# Autodesk Inventor assembly: 110033226_iam_10_角落碉堡
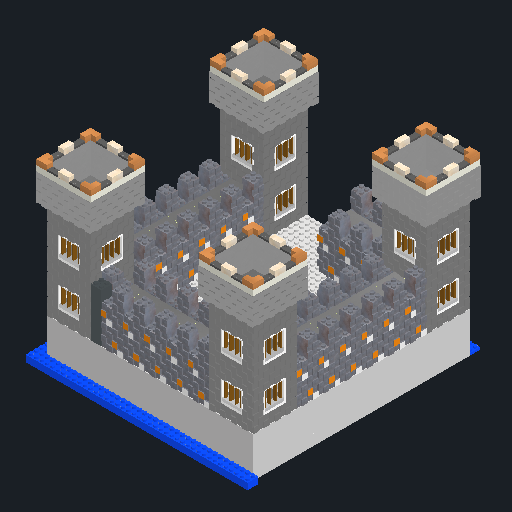
[picture p0: Inventor's stored thumbnail of the model, 512x512]
Saved by Autodesk Inventor 2022 (Build 260153000, 153)
## iProperties
Created: 2022-06-28
Part Number: 110033226_iam_10_角落碉堡
Document SubType Name: Assembly
Designer: User
Author: User
## Documents named in this file (6)
- D:\D-disk\pomelo\大一\下學期\機械設計製圖\1100332260_LEGOproj_沒有公主城堡\110033226_iam_10_角落碉堡.iam
- D:\D-disk\pomelo\大一\下學期\機械設計製圖\1100332260_LEGOproj_沒有公主城堡\110033226_ipt_43_角落碉堡基座.ipt
- D:\D-disk\pomelo\大一\下學期\機械設計製圖\1100332260_LEGOproj_沒有公主城堡\110033226_ipt_04_小河.ipt
- D:\D-disk\pomelo\大一\下學期\機械設計製圖\1100332260_LEGOproj_沒有公主城堡\110033226_iam_06_城堡四角塔.iam
- D:\D-disk\pomelo\大一\下學期\機械設計製圖\1100332260_LEGOproj_沒有公主城堡\110033226_ipt_34_中心城堡圍牆.ipt
- D:\D-disk\pomelo\大一\下學期\機械設計製圖\1100332260_LEGOproj_沒有公主城堡\110033226_ipt_24_直條(3x1).ipt
## Components (158 placed, 5 different names)
1. 110033226_ipt_34_中心城堡圍牆:39 — 貼合:27, 貼合:28, 貼合:29, 貼合:38
2. 110033226_ipt_43_角落碉堡基座:1 — 貼合:1, 貼合:2, 貼合:3, 貼合:4, 貼合:5, 貼合:6, 貼合:7, 貼合:8, 貼合:9, 貼合:11
3. 110033226_ipt_43_角落碉堡基座:2
4. 110033226_ipt_43_角落碉堡基座:3
5. 110033226_ipt_43_角落碉堡基座:4
6. 110033226_ipt_43_角落碉堡基座:5
7. 110033226_ipt_43_角落碉堡基座:6
8. 110033226_ipt_43_角落碉堡基座:7
9. 110033226_ipt_43_角落碉堡基座:8
10. 110033226_ipt_43_角落碉堡基座:9
11. 110033226_ipt_43_角落碉堡基座:10
12. 110033226_ipt_43_角落碉堡基座:11
13. 110033226_ipt_43_角落碉堡基座:12
14. 110033226_ipt_43_角落碉堡基座:13
15. 110033226_ipt_43_角落碉堡基座:14
16. 110033226_ipt_43_角落碉堡基座:15 — 貼合:12, 貼合:13, 貼合:14, 貼合:15, 貼合:16, 貼合:17, 貼合:18, 貼合:19, 貼合:21, 貼合:22, 貼合:23, 貼合:24, 貼合:25, 貼合:26, 貼合:27, 貼合:28, 貼合:29, 貼合:30, 貼合:31, 貼合:32, 貼合:33, 貼合:34, 貼合:35, 貼合:36, 貼合:37
17. 110033226_ipt_04_小河:4 — 貼合:7, 貼合:8, 貼合:9
18. 110033226_ipt_04_小河:5
19. 110033226_ipt_04_小河:6
20. 110033226_ipt_04_小河:7
21. 110033226_ipt_04_小河:8
22. 110033226_ipt_04_小河:9
23. 110033226_ipt_04_小河:10
24. 110033226_ipt_04_小河:11
25. 110033226_ipt_04_小河:12
26. 110033226_ipt_04_小河:13
27. 110033226_ipt_04_小河:14
28. 110033226_ipt_04_小河:15
29. 110033226_ipt_04_小河:16
30. 110033226_ipt_04_小河:17
31. 110033226_ipt_04_小河:18
32. 110033226_ipt_04_小河:19
33. 110033226_ipt_04_小河:20
34. 110033226_ipt_04_小河:21
35. 110033226_ipt_04_小河:22
36. 110033226_ipt_04_小河:23
37. 110033226_ipt_04_小河:24
38. 110033226_ipt_04_小河:25
39. 110033226_ipt_04_小河:26
40. 110033226_ipt_04_小河:27
41. 110033226_ipt_04_小河:28
42. 110033226_ipt_04_小河:29
43. 110033226_ipt_04_小河:30
44. 110033226_ipt_04_小河:31
45. 110033226_ipt_04_小河:32
46. 110033226_ipt_04_小河:33
47. 110033226_ipt_04_小河:34
48. 110033226_ipt_04_小河:35
49. 110033226_ipt_04_小河:36
50. 110033226_ipt_04_小河:37
51. 110033226_ipt_04_小河:38
52. 110033226_ipt_04_小河:39
53. 110033226_ipt_04_小河:40
54. 110033226_ipt_04_小河:41
55. 110033226_ipt_04_小河:42
56. 110033226_ipt_04_小河:43 — 對稱:1, 貼合:10
57. 110033226_ipt_04_小河:44
58. 110033226_ipt_04_小河:45
59. 110033226_ipt_04_小河:3 — 對稱:1, 貼合:10, 貼合:11
60. 110033226_ipt_04_小河:46
61. 110033226_ipt_04_小河:47
62. 110033226_ipt_04_小河:48
63. 110033226_ipt_04_小河:49
64. 110033226_ipt_04_小河:50
65. 110033226_ipt_04_小河:51
66. 110033226_ipt_04_小河:52
67. 110033226_ipt_04_小河:53
68. 110033226_ipt_04_小河:54
69. 110033226_ipt_04_小河:55
70. 110033226_ipt_04_小河:56
71. 110033226_ipt_04_小河:57
72. 110033226_ipt_04_小河:58
73. 110033226_ipt_04_小河:59
74. 110033226_ipt_04_小河:60
75. 110033226_ipt_04_小河:61
76. 110033226_ipt_04_小河:62
77. 110033226_ipt_04_小河:63
78. 110033226_ipt_04_小河:64
79. 110033226_ipt_04_小河:65
80. 110033226_ipt_04_小河:66
81. 110033226_ipt_04_小河:67
82. 110033226_ipt_04_小河:68
83. 110033226_ipt_04_小河:69
84. 110033226_ipt_04_小河:70
85. 110033226_ipt_04_小河:71
86. 110033226_ipt_04_小河:72
87. 110033226_ipt_04_小河:73
88. 110033226_ipt_04_小河:74
89. 110033226_ipt_04_小河:75
90. 110033226_ipt_04_小河:76
91. 110033226_ipt_04_小河:77
92. 110033226_ipt_04_小河:78
93. 110033226_ipt_04_小河:79
94. 110033226_ipt_04_小河:80
95. 110033226_ipt_04_小河:81
96. 110033226_ipt_04_小河:82
97. 110033226_ipt_04_小河:83
98. 110033226_ipt_04_小河:1 — 貼合:4, 貼合:5, 貼合:6
99. 110033226_ipt_04_小河:84
100. 110033226_ipt_04_小河:85
101. 110033226_ipt_04_小河:86
102. 110033226_ipt_04_小河:87
103. 110033226_iam_06_城堡四角塔:1 [sub-assembly] — 貼合:12, 貼合:13, 貼合:14
104. 110033226_iam_06_城堡四角塔:2 [sub-assembly]
105. 110033226_iam_06_城堡四角塔:3 [sub-assembly]
106. 110033226_iam_06_城堡四角塔:4 [sub-assembly]
107. 110033226_ipt_34_中心城堡圍牆:3 — 貼合:18, 貼合:19, 貼合:20
108. 110033226_ipt_34_中心城堡圍牆:1 — 貼合:15, 貼合:16, 貼合:17, 貼合:20
109. 110033226_ipt_34_中心城堡圍牆:5
110. 110033226_ipt_34_中心城堡圍牆:6
111. 110033226_ipt_34_中心城堡圍牆:7
112. 110033226_ipt_34_中心城堡圍牆:8
113. 110033226_ipt_34_中心城堡圍牆:9
114. 110033226_ipt_34_中心城堡圍牆:10
115. 110033226_ipt_34_中心城堡圍牆:11
116. 110033226_ipt_34_中心城堡圍牆:12
117. 110033226_ipt_34_中心城堡圍牆:13
118. 110033226_ipt_34_中心城堡圍牆:14
119. 110033226_ipt_34_中心城堡圍牆:15
120. 110033226_ipt_34_中心城堡圍牆:16
121. 110033226_ipt_34_中心城堡圍牆:17
122. 110033226_ipt_34_中心城堡圍牆:18
123. 110033226_ipt_34_中心城堡圍牆:19
124. 110033226_ipt_34_中心城堡圍牆:20
125. 110033226_ipt_34_中心城堡圍牆:21
126. 110033226_ipt_34_中心城堡圍牆:22
127. 110033226_ipt_34_中心城堡圍牆:23
128. 110033226_ipt_34_中心城堡圍牆:24
129. 110033226_ipt_34_中心城堡圍牆:25
130. 110033226_ipt_34_中心城堡圍牆:26
131. 110033226_ipt_34_中心城堡圍牆:28 — 貼合:25, 齊平:1, 貼合:26
132. 110033226_ipt_34_中心城堡圍牆:27 — 貼合:21, 貼合:22, 貼合:23, 貼合:24, 齊平:1
133. 110033226_ipt_34_中心城堡圍牆:29
134. 110033226_ipt_34_中心城堡圍牆:30
135. 110033226_ipt_34_中心城堡圍牆:31
136. 110033226_ipt_34_中心城堡圍牆:32
137. 110033226_ipt_34_中心城堡圍牆:33
138. 110033226_ipt_34_中心城堡圍牆:34
139. 110033226_ipt_34_中心城堡圍牆:35
140. 110033226_ipt_34_中心城堡圍牆:36
141. 110033226_ipt_34_中心城堡圍牆:37
142. 110033226_ipt_34_中心城堡圍牆:38
143. 110033226_ipt_34_中心城堡圍牆:41 — 貼合:33, 貼合:34, 貼合:35
144. 110033226_ipt_34_中心城堡圍牆:40 — 貼合:30, 貼合:31, 貼合:32
145. 110033226_ipt_34_中心城堡圍牆:42
146. 110033226_ipt_34_中心城堡圍牆:43
147. 110033226_ipt_24_直條(3x1):1 — 貼合:36, 貼合:37, 貼合:38
148. 110033226_ipt_24_直條(3x1):2
149. 110033226_ipt_24_直條(3x1):3
150. 110033226_ipt_24_直條(3x1):4
151. 110033226_ipt_24_直條(3x1):5
152. 110033226_ipt_24_直條(3x1):6
153. 110033226_ipt_24_直條(3x1):7
154. 110033226_ipt_24_直條(3x1):8
155. 110033226_ipt_24_直條(3x1):9
156. 110033226_ipt_24_直條(3x1):10
157. 110033226_ipt_24_直條(3x1):11
158. 110033226_ipt_24_直條(3x1):12
## Component patterns: (15 elements, first: 110033226_ipt_43_角落碉堡基座:1), (42 elements, first: 110033226_ipt_04_小河:4), (39 elements, first: 110033226_ipt_04_小河:3), (5 elements, first: 110033226_ipt_04_小河:1), (4 elements, first: 110033226_iam_06_城堡四角塔:1), (12 elements, first: 110033226_ipt_34_中心城堡圍牆:3 + 110033226_ipt_34_中心城堡圍牆:1), (6 elements, first: 110033226_ipt_34_中心城堡圍牆:28 + 110033226_ipt_34_中心城堡圍牆:27), (2 elements, first: 110033226_ipt_34_中心城堡圍牆:41 + 110033226_ipt_34_中心城堡圍牆:40), (3 elements), (4 elements, first: 110033226_ipt_24_直條(3x1):1), 元件陣列 11:2 (4 elements), 元件陣列 11:3 (4 elements)
## Relationships (40: Mate 38, Symmetry 1, Flush 1)
- 貼合:1 [Mate]: 110033226_ipt_43_角落碉堡基座:1
- 貼合:2 [Mate]: 110033226_ipt_43_角落碉堡基座:1
- 貼合:3 [Mate]: 110033226_ipt_43_角落碉堡基座:1
- 貼合:4 [Mate]: 110033226_ipt_43_角落碉堡基座:1 ↔ 110033226_ipt_04_小河:1
- 貼合:5 [Mate]: 110033226_ipt_43_角落碉堡基座:1 ↔ 110033226_ipt_04_小河:1
- 貼合:6 [Mate]: 110033226_ipt_43_角落碉堡基座:1 ↔ 110033226_ipt_04_小河:1
- 貼合:7 [Mate]: 110033226_ipt_43_角落碉堡基座:1 ↔ 110033226_ipt_04_小河:4
- 貼合:8 [Mate]: 110033226_ipt_43_角落碉堡基座:1 ↔ 110033226_ipt_04_小河:4
- 貼合:9 [Mate]: 110033226_ipt_43_角落碉堡基座:1 ↔ 110033226_ipt_04_小河:4
- 對稱:1 [Symmetry]: 110033226_ipt_04_小河:43 ↔ 110033226_ipt_04_小河:3
- 貼合:10 [Mate]: 110033226_ipt_04_小河:43 ↔ 110033226_ipt_04_小河:3
- 貼合:11 [Mate]: 110033226_ipt_43_角落碉堡基座:1 ↔ 110033226_ipt_04_小河:3
- 貼合:12 [Mate]: 110033226_ipt_43_角落碉堡基座:15 ↔ 110033226_iam_06_城堡四角塔:1
- 貼合:13 [Mate]: 110033226_ipt_43_角落碉堡基座:15 ↔ 110033226_iam_06_城堡四角塔:1
- 貼合:14 [Mate]: 110033226_ipt_43_角落碉堡基座:15 ↔ 110033226_iam_06_城堡四角塔:1
- 貼合:15 [Mate]: 110033226_ipt_43_角落碉堡基座:15 ↔ 110033226_ipt_34_中心城堡圍牆:1
- 貼合:16 [Mate]: 110033226_ipt_43_角落碉堡基座:15 ↔ 110033226_ipt_34_中心城堡圍牆:1
- 貼合:17 [Mate]: 110033226_ipt_43_角落碉堡基座:15 ↔ 110033226_ipt_34_中心城堡圍牆:1
- 貼合:18 [Mate]: 110033226_ipt_43_角落碉堡基座:15 ↔ 110033226_ipt_34_中心城堡圍牆:3
- 貼合:19 [Mate]: 110033226_ipt_43_角落碉堡基座:15 ↔ 110033226_ipt_34_中心城堡圍牆:3
- 貼合:20 [Mate]: 110033226_ipt_34_中心城堡圍牆:3 ↔ 110033226_ipt_34_中心城堡圍牆:1
- 貼合:21 [Mate]: 110033226_ipt_43_角落碉堡基座:15 ↔ 110033226_ipt_34_中心城堡圍牆:27
- 貼合:22 [Mate]: 110033226_ipt_43_角落碉堡基座:15 ↔ 110033226_ipt_34_中心城堡圍牆:27
- 貼合:23 [Mate]: 110033226_ipt_43_角落碉堡基座:15 ↔ 110033226_ipt_34_中心城堡圍牆:27
- 貼合:24 [Mate]: 110033226_ipt_43_角落碉堡基座:15 ↔ 110033226_ipt_34_中心城堡圍牆:27
- 貼合:25 [Mate]: 110033226_ipt_43_角落碉堡基座:15 ↔ 110033226_ipt_34_中心城堡圍牆:28
- 齊平:1 [Flush]: 110033226_ipt_34_中心城堡圍牆:28 ↔ 110033226_ipt_34_中心城堡圍牆:27
- 貼合:26 [Mate]: 110033226_ipt_43_角落碉堡基座:15 ↔ 110033226_ipt_34_中心城堡圍牆:28
- 貼合:27 [Mate]: 110033226_ipt_34_中心城堡圍牆:39 ↔ 110033226_ipt_43_角落碉堡基座:15
- 貼合:28 [Mate]: 110033226_ipt_34_中心城堡圍牆:39 ↔ 110033226_ipt_43_角落碉堡基座:15
- 貼合:29 [Mate]: 110033226_ipt_34_中心城堡圍牆:39 ↔ 110033226_ipt_43_角落碉堡基座:15
- 貼合:30 [Mate]: 110033226_ipt_43_角落碉堡基座:15 ↔ 110033226_ipt_34_中心城堡圍牆:40
- 貼合:31 [Mate]: 110033226_ipt_43_角落碉堡基座:15 ↔ 110033226_ipt_34_中心城堡圍牆:40
- 貼合:32 [Mate]: 110033226_ipt_43_角落碉堡基座:15 ↔ 110033226_ipt_34_中心城堡圍牆:40
- 貼合:33 [Mate]: 110033226_ipt_43_角落碉堡基座:15 ↔ 110033226_ipt_34_中心城堡圍牆:41
- 貼合:34 [Mate]: 110033226_ipt_43_角落碉堡基座:15 ↔ 110033226_ipt_34_中心城堡圍牆:41
- 貼合:35 [Mate]: 110033226_ipt_43_角落碉堡基座:15 ↔ 110033226_ipt_34_中心城堡圍牆:41
- 貼合:36 [Mate]: 110033226_ipt_43_角落碉堡基座:15 ↔ 110033226_ipt_24_直條(3x1):1
- 貼合:37 [Mate]: 110033226_ipt_43_角落碉堡基座:15 ↔ 110033226_ipt_24_直條(3x1):1
- 貼合:38 [Mate]: 110033226_ipt_34_中心城堡圍牆:39 ↔ 110033226_ipt_24_直條(3x1):1
